# Autodesk Inventor assembly: MG_996R
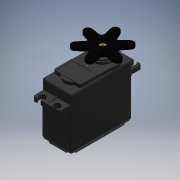
[picture p0: Inventor's stored thumbnail of the model, 180x180]
Saved by Autodesk Inventor 2019 (Build 230136000, 136)
## iProperties
Created: 2016-09-26
Part Number: MG_996R
Document SubType Name: Assembly
Designer: Julian
Author: Julian
## Documents named in this file (7)
- C:\Users\jacqu\Desktop\Robotica1_Proyecto-Cuadrupedo-master\Robotica1-Proyecto_Cuadrupedo\MG_996R.iam
- C:\Users\jacqu\Desktop\Robotica1_Proyecto-Cuadrupedo-master\Robotica1-Proyecto_Cuadrupedo\Base.ipt
- C:\Users\jacqu\Desktop\Robotica1_Proyecto-Cuadrupedo-master\Robotica1-Proyecto_Cuadrupedo\Medio.ipt
- C:\Users\jacqu\Desktop\Robotica1_Proyecto-Cuadrupedo-master\Robotica1-Proyecto_Cuadrupedo\Top.ipt
- C:\Users\jacqu\Desktop\Robotica1_Proyecto-Cuadrupedo-master\Robotica1-Proyecto_Cuadrupedo\Eje.ipt
- C:\Users\jacqu\Desktop\Robotica1_Proyecto-Cuadrupedo-master\Robotica1-Proyecto_Cuadrupedo\Acople circular.ipt
- C:\Users\jacqu\Desktop\Robotica1_Proyecto-Cuadrupedo-master\Robotica1-Proyecto_Cuadrupedo\Sevo arm TowerPro SG-5010.ipt
## Components (6 placed, 6 different names)
1. Top:1 — Rígido:2, De rotación:1, Mate:1
2. Medio:1 — Rígido:1, Rígido:2
3. Base:1 — Rígido:1
4. Eje:1 — De rotación:1, De rotación:2, Mate:2
5. Acople circular:1 — De rotación:2
6. Sevo arm TowerPro SG-5010:1 — Mate:1, Mate:2
## Relationships (6: WeldJoint 2, RevoluteJoint 2, Mate 2)
- Rígido:1 [WeldJoint]: Medio:1 ↔ Base:1
- Rígido:2 [WeldJoint]: Top:1 ↔ Medio:1
- De rotación:1 [RevoluteJoint]: Top:1 ↔ Eje:1
- De rotación:2 [RevoluteJoint]: Eje:1 ↔ Acople circular:1
- Mate:1 (3.3 mm): Top:1 ↔ Sevo arm TowerPro SG-5010:1
- Mate:2: Eje:1 ↔ Sevo arm TowerPro SG-5010:1
